# Autodesk Inventor assembly: Assembly
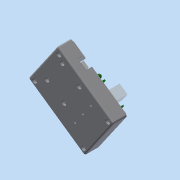
[picture p0: Inventor's stored thumbnail of the model, 180x180]
Saved by Autodesk Inventor 2015 (Build 190159000, 159)
## iProperties
Created: 2014-12-25
Part Number: Assembly
Document SubType Name: Assembly
Designer: Openlab
Author: Openlab
## Documents named in this file (9)
- C:\Users\Openlab\Documents\Alexey\HS-Spectrophotometer\parts\Assembly.iam
- C:\Users\Openlab\Documents\Alexey\HS-Spectrophotometer\parts\Motherboard_dummy.ipt
- C:\Users\Openlab\Documents\Alexey\HS-Spectrophotometer\parts\Sensor_Board_dummy.ipt
- C:\Users\Openlab\Documents\Alexey\HS-Spectrophotometer\parts\Led_Board_V1.ipt
- C:\Users\Openlab\Documents\Alexey\HS-Spectrophotometer\parts\filter.ipt
- C:\Users\Openlab\Documents\Alexey\HS-Spectrophotometer\parts\Base_V2.ipt
- C:\Users\Openlab\Documents\Alexey\HS-Spectrophotometer\parts\TopV2.ipt
- C:\Users\Openlab\Documents\Alexey\HS-Spectrophotometer\parts\Cover.ipt
- C:\Users\Openlab\Documents\Alexey\HS-Spectrophotometer\parts\Cuvette.ipt
## Components (9 placed, 8 different names)
1. Motherboard_dummy:1 — Mate:1, Mate:2, Mate:3
2. Sensor_Board_dummy:1 — Mate:7, Mate:8, Mate:9
3. Led_Board_V1:1 — Mate:4, Mate:5, Mate:6
4. filter:1 — Mate:10, Mate:11, Mate:12
5. filter:2 — Mate:13, Mate:14, Mate:15
6. Base_V2:1 — Mate:1, Mate:2, Mate:3, Mate:4, Mate:5, Mate:6, Mate:7, Mate:8, Mate:9, Mate:10, Mate:11, Mate:12, Mate:13, Mate:14, Mate:15, Mate:17, Mate:18, Mate:22, Mate:23, Mate:24, Mate:25, Mate:26, Mate:27, Mate:28
7. TopV2:1 — Mate:17, Mate:18, Mate:19, Mate:20, Mate:21, Mate:25, Mate:26, Mate:27, Mate:28, Mate:29, Mate:30, Mate:31
8. Cover:1 — Mate:19, Mate:20, Mate:21, Mate:29, Mate:30, Mate:31
9. Cuvette:1 — Mate:22, Mate:23, Mate:24
## Relationships (30: Mate 30)
- Mate:1: Motherboard_dummy:1 ↔ Base_V2:1
- Mate:2: Motherboard_dummy:1 ↔ Base_V2:1
- Mate:3: Motherboard_dummy:1 ↔ Base_V2:1
- Mate:4: Led_Board_V1:1 ↔ Base_V2:1
- Mate:5: Led_Board_V1:1 ↔ Base_V2:1
- Mate:6: Led_Board_V1:1 ↔ Base_V2:1
- Mate:7: Sensor_Board_dummy:1 ↔ Base_V2:1
- Mate:8: Sensor_Board_dummy:1 ↔ Base_V2:1
- Mate:9: Sensor_Board_dummy:1 ↔ Base_V2:1
- Mate:10: filter:1 ↔ Base_V2:1
- Mate:11: filter:1 ↔ Base_V2:1
- Mate:12: filter:1 ↔ Base_V2:1
- Mate:13: filter:2 ↔ Base_V2:1
- Mate:14: filter:2 ↔ Base_V2:1
- Mate:15: filter:2 ↔ Base_V2:1
- Mate:17: Base_V2:1 ↔ TopV2:1
- Mate:18: Base_V2:1 ↔ TopV2:1
- Mate:19: TopV2:1 ↔ Cover:1
- Mate:20: TopV2:1 ↔ Cover:1
- Mate:21: TopV2:1 ↔ Cover:1
- Mate:22: Base_V2:1 ↔ Cuvette:1
- Mate:23: Base_V2:1 ↔ Cuvette:1
- Mate:24: Base_V2:1 ↔ Cuvette:1
- Mate:25: Base_V2:1 ↔ TopV2:1
- Mate:26: Base_V2:1 ↔ TopV2:1
- Mate:27: Base_V2:1 ↔ TopV2:1
- Mate:28: Base_V2:1 ↔ TopV2:1
- Mate:29: TopV2:1 ↔ Cover:1
- Mate:30: TopV2:1 ↔ Cover:1
- Mate:31: TopV2:1 ↔ Cover:1
